# Autodesk Inventor assembly: Frame0001
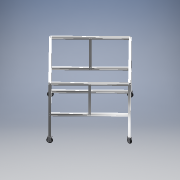
[picture p0: Inventor's stored thumbnail of the model, 180x180]
Saved by Autodesk Inventor 2019 (Build 230136000, 136)
## iProperties
Created: 2019-11-22
Part Number: Frame0001
Document SubType Name: Assembly
Designer: felix
Mass: 47055.5 g
Surface Area: 67197.3 cm^2
Volume: 15566 cm^3
Density: 3.02296 g/cm^3
_FrameDoc: Frame Assembly
_Version: 15.0.0
Author: felix
## Documents named in this file (39)
- D:\Downloads\RuedaGiratoria\Frame\Frame0001.iam
- D:\Downloads\RuedaGiratoria\Frame\Skeleton0001.ipt
- D:\Documents\Inventor\Content Center Files\R2019\en-US\AS 1420\AS 1420 - 1973 - M6 x 25.ipt
- D:\Downloads\castor-wheel-4-1.snapshot.1\CASTOR 4\Castor 4.iam
- D:\Documents\Inventor\Content Center Files\R2019\en-US\AS 1420\AS 1420 - 1973 - M6 x 12.ipt
- D:\Downloads\RuedaGiratoria\Frame\FEL2  00000048.ipt
- FEL2  00000048.ipt
- D:\Downloads\RuedaGiratoria\Frame\FEL2  00000049.ipt
- FEL2  00000049.ipt
- D:\Downloads\RuedaGiratoria\Frame\FEL2  00000050.ipt
- FEL2  00000050.ipt
- D:\Downloads\RuedaGiratoria\Frame\FEL2  00000051.ipt
- FEL2  00000051.ipt
- D:\Downloads\RuedaGiratoria\Frame\FEL2  00000052.ipt
- FEL2  00000052.ipt
- D:\Downloads\RuedaGiratoria\Frame\FEL2  00000053.ipt
- FEL2  00000053.ipt
- D:\Downloads\RuedaGiratoria\Frame\FEL2  00000054.ipt
- FEL2  00000054.ipt
- D:\Downloads\RuedaGiratoria\Frame\FEL2  00000055.ipt
- FEL2  00000055.ipt
- D:\Downloads\RuedaGiratoria\Frame\FEL2  00000056.ipt
- FEL2  00000056.ipt
- D:\Downloads\RuedaGiratoria\Frame\FEL2  00000057.ipt
- FEL2  00000057.ipt
- D:\Downloads\RuedaGiratoria\Frame\FEL2  00000058.ipt
- FEL2  00000058.ipt
- D:\Downloads\RuedaGiratoria\Frame\FEL2  00000059.ipt
- FEL2  00000059.ipt
- D:\Downloads\RuedaGiratoria\Frame\FEL2  00000060.ipt
- FEL2  00000060.ipt
- D:\Downloads\RuedaGiratoria\Frame\FEL2  00000061.ipt
- FEL2  00000061.ipt
- D:\Downloads\RuedaGiratoria\Frame\FEL2  00000062.ipt
- FEL2  00000062.ipt
- D:\Downloads\RuedaGiratoria\Frame\FEL2  00000063.ipt
- FEL2  00000063.ipt
- D:\Downloads\RuedaGiratoria\Frame\FEL2  00000064.ipt
- FEL2  00000064.ipt
## Components (30 placed, 21 different names)
1. Frame Reference Model
2. AS 1420 - Metric M6 x 25:1
3. Castor 4:1 [sub-assembly] — Mate:19, Mate:20
4. Castor 4:2 [sub-assembly] — Mate:21, Mate:22
5. Castor 4:3 [sub-assembly] — Mate:23, Mate:24
6. Castor 4:4 [sub-assembly] — Mate:18
7. AS 1420 - Metric M6 x 25:2
8. AS 1420 - Metric M6 x 25:3
9. AS 1420 - Metric M6 x 25:4
10. AS 1420 - Metric M6 x 12:1 — Mate:18
11. AS 1420 - Metric M6 x 12:2 — Mate:19, Mate:20
12. AS 1420 - Metric M6 x 12:3 — Mate:21, Mate:22
13. AS 1420 - Metric M6 x 12:4 — Mate:23, Mate:24
14. FEL2  00000048:1
15. FEL2  00000049:1
16. FEL2  00000050:1
17. FEL2  00000051:1
18. FEL2  00000052:1
19. FEL2  00000053:1
20. FEL2  00000054:1
21. FEL2  00000055:1
22. FEL2  00000056:1
23. FEL2  00000057:1
24. FEL2  00000058:1
25. FEL2  00000059:1
26. FEL2  00000060:1
27. FEL2  00000061:1
28. FEL2  00000062:1
29. FEL2  00000063:1
30. FEL2  00000064:1
## Relationships (7: Mate 7)
- Mate:18: Castor 4:4 ↔ AS 1420 - Metric M6 x 12:1
- Mate:19: Castor 4:1 ↔ AS 1420 - Metric M6 x 12:2
- Mate:20: Castor 4:1 ↔ AS 1420 - Metric M6 x 12:2
- Mate:21: Castor 4:2 ↔ AS 1420 - Metric M6 x 12:3
- Mate:22: Castor 4:2 ↔ AS 1420 - Metric M6 x 12:3
- Mate:23: Castor 4:3 ↔ AS 1420 - Metric M6 x 12:4
- Mate:24: Castor 4:3 ↔ AS 1420 - Metric M6 x 12:4
